# Autodesk Inventor assembly: Arduino uno r3
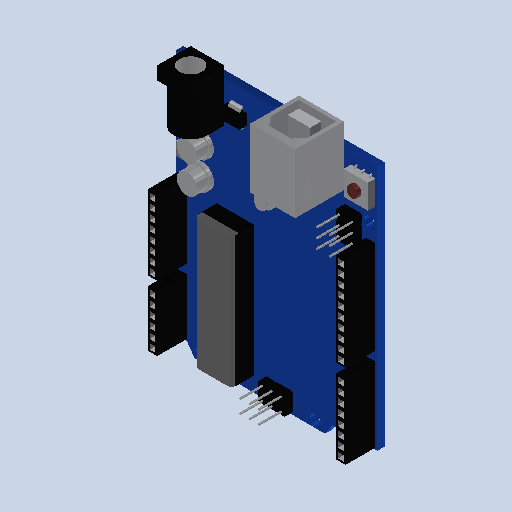
[picture p0: Inventor's stored thumbnail of the model, 512x512]
Saved by Autodesk Inventor 2022 (Build 260153000, 153)
## iProperties
Created: 2017-06-03
Part Number: Arduino uno r3
Document SubType Name: Assembly
Designer: L.Đ.P
Mass: 13.5145 g
Surface Area: 153.784 cm^2
Volume: 13.5632 cm^3
Density: 0.996411 g/cm^3
Author: L.Đ.P
## Documents named in this file (3)
- C:\Users\JK\Documents\Inventor\UTM\Arduino uno r3.iam
- C:\Users\JK\Documents\Inventor\UTM\Arduino UNO R3.ipt
- C:\Users\JK\Documents\Inventor\UTM\ATMEGA328P-PV.ipt
## Components (2 placed, 2 different names)
1. Arduino UNO R3:1 — Flush:1, Flush:2, Mate:1
2. ATMEGA328P-PV:1 — Flush:1, Flush:2, Mate:1
## Relationships (3: Flush 2, Mate 1)
- Flush:1: Arduino UNO R3:1 ↔ ATMEGA328P-PV:1
- Flush:2: Arduino UNO R3:1 ↔ ATMEGA328P-PV:1
- Mate:1: Arduino UNO R3:1 ↔ ATMEGA328P-PV:1
